# Autodesk Inventor assembly: 90mm dual omni wheels
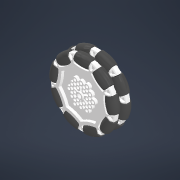
[picture p0: Inventor's stored thumbnail of the model, 180x180]
Saved by Autodesk Inventor 2022 (Build 260153000, 153)
## iProperties
Created: 2021-09-18
Part Number: 90mm dual omni wheels
Document SubType Name: Assembly
Designer: izack
Author: izack
## Documents named in this file (2)
- D:\Robotics\ComputerAidedDesign\2021-22\FTC\#13822 Robovikes\Proof of Concept\90mm dual omni wheels.iam
- D:\Robotics\ComputerAidedDesign\2021-22\FTC\#13822 Robovikes\Proof of Concept\90mm Omni Wheel - 2 Pack.ipt
## Components (2 placed, 1 different names)
1. 90mm Omni Wheel - 2 Pack:1 — Flush:1, Flush:2, Mate:1
2. 90mm Omni Wheel - 2 Pack:2 — Flush:1, Flush:2, Mate:1
## Relationships (3: Flush 2, Mate 1)
- Flush:1: 90mm Omni Wheel - 2 Pack:1 ↔ 90mm Omni Wheel - 2 Pack:2
- Flush:2: 90mm Omni Wheel - 2 Pack:1 ↔ 90mm Omni Wheel - 2 Pack:2
- Mate:1: 90mm Omni Wheel - 2 Pack:1 ↔ 90mm Omni Wheel - 2 Pack:2
